# Autodesk Inventor assembly: OBG-Kicker
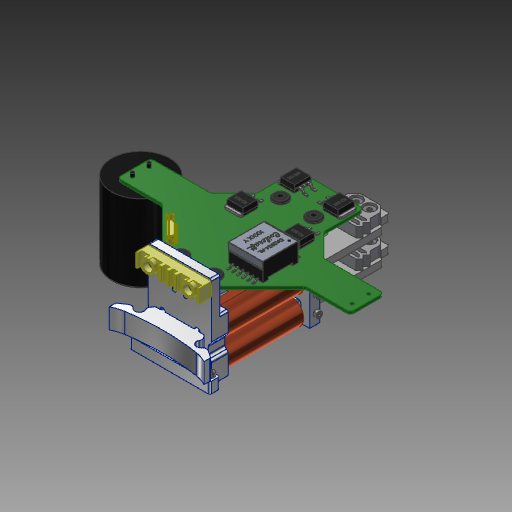
[picture p0: Inventor's stored thumbnail of the model, 512x512]
Saved by Autodesk Inventor 2019.4 (Build 234330000, 330)
## iProperties
Part Number: OBG-Kicker
Material: Generisch
Document SubType Name: Assembly
Designer: rYan
Mass: 621.618 g
Surface Area: 1033.16 cm^2
Volume: 199.876 cm^3
Density: 3.11002 g/cm^3
Author: rYan
## Documents named in this file (6)
- D:\TIGERsGIT\Hardware\mechanik\2020\Inventor\Robot\Kicker\OBG-Kicker.iam
- D:\TIGERsGIT\Hardware\mechanik\2020\Inventor\Robot\Kicker\UBG-Spulen.iam
- D:\TIGERsGIT\Hardware\mechanik\2020\Inventor\Robot\Kicker\MG-Chip Kicker.iam
- D:\TIGERsGIT\Hardware\mechanik\2020\Inventor\Robot\Kicker\MG-Straight Kicker.iam
- D:\TIGERsGIT\Hardware\mechanik\2020\Inventor\Robot\Electronics\MG-Kickerboard.iam
- D:\TIGERsGIT\Hardware\mechanik\2020\Inventor\Inhaltscenter\de-DE\ISO 10642(1)\ISO 10642 - M3 x  8.ipt
## Components (8 placed, 5 different names)
1. UBG-Spulen:1 [sub-assembly] — Fluchtend:1, Fluchtend:2, Fluchtend:3, Passend:5, Passend:6, Passend:7, Passend:8, Passend:9, Passend:10, Passend:11
2. MG-Chip Kicker:1 [sub-assembly] — Passend:1, Passend:9, Passend:11
3. MG-Straight Kicker:1 [sub-assembly] — Passend:3, Passend:8, Passend:10
4. MG-Kickerboard:1 [sub-assembly] — Passend:5, Passend:6, Passend:7, Einfügen:1, Einfügen:2, Einfügen:3, Einfügen:4
5. ISO 10642 M3 x  8:1 — Einfügen:1
6. ISO 10642 M3 x  8:2 — Einfügen:2
7. ISO 10642 M3 x  8:3 — Einfügen:3
8. ISO 10642 M3 x  8:4 — Einfügen:4
## Relationships (16: Mate 9, Insert 4, Flush 3)
- Fluchtend:1 [Flush]: UBG-Spulen:1
- Fluchtend:2 [Flush]: UBG-Spulen:1
- Fluchtend:3 [Flush]: UBG-Spulen:1
- Passend:1 [Mate]: MG-Chip Kicker:1
- Passend:3 [Mate]: MG-Straight Kicker:1
- Passend:5 [Mate]: UBG-Spulen:1 ↔ MG-Kickerboard:1
- Passend:6 [Mate]: UBG-Spulen:1 ↔ MG-Kickerboard:1
- Passend:7 [Mate]: UBG-Spulen:1 ↔ MG-Kickerboard:1
- Passend:8 [Mate] (0.05 mm): UBG-Spulen:1 ↔ MG-Straight Kicker:1
- Passend:9 [Mate] (0.05 mm): UBG-Spulen:1 ↔ MG-Chip Kicker:1
- Passend:10 [Mate]: UBG-Spulen:1 ↔ MG-Straight Kicker:1
- Passend:11 [Mate]: UBG-Spulen:1 ↔ MG-Chip Kicker:1
- Einfügen:1 [Insert] (-0.5 mm): MG-Kickerboard:1 ↔ ISO 10642 M3 x  8:1
- Einfügen:2 [Insert] (-0.5 mm): MG-Kickerboard:1 ↔ ISO 10642 M3 x  8:2
- Einfügen:3 [Insert] (-0.5 mm): MG-Kickerboard:1 ↔ ISO 10642 M3 x  8:3
- Einfügen:4 [Insert] (-0.5 mm): MG-Kickerboard:1 ↔ ISO 10642 M3 x  8:4
